# Autodesk Inventor assembly: Assembly_for_print
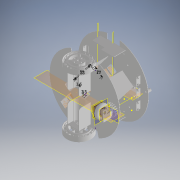
[picture p0: Inventor's stored thumbnail of the model, 180x180]
Saved by Autodesk Inventor 2020 (Build 240168000, 168)
## iProperties
Created: 2020-10-03
Part Number: Assembly_for_print
Document SubType Name: Assembly
Designer: Sičaja
Author: Sičaja
## Documents named in this file (7)
- C:\Users\Sicaja\Documents\Projects\3D Drawings\Inventor_draws\Robocup\Inverntor_parts_for_print\Assembly_for_print.iam
- C:\Users\Sicaja\Documents\Projects\3D Drawings\Inventor_draws\Robocup\Inverntor_parts_for_print\DropMechanism_v.2.0.ipt
- C:\Users\Sicaja\Documents\Projects\3D Drawings\Inventor_draws\Robocup\Inverntor_parts_for_print\KonstrukcijaDonjiDio_v.1.1.ipt
- C:\Users\Sicaja\Documents\Projects\3D Drawings\Inventor_draws\Robocup\Inverntor_parts_for_print\Gornja_konstrukcija_s_držačima_assembly_converted.ipt
- C:\Users\Sicaja\Documents\Projects\3D Drawings\Inventor_draws\Robocup\Inverntor_parts_for_print\Kotač_v.2.0.ipt
- C:\Users\Sicaja\Documents\Projects\3D Drawings\Inventor_draws\Robocup\Inverntor_parts_for_print\DrzacZaPrednjiKotač_v.1.0.ipt
- C:\Users\Sicaja\Documents\Projects\3D Drawings\Inventor_draws\Robocup\Inverntor_parts_for_print\PrednjiKotač_635z_lezaj_v.2.0.ipt
## Components (7 placed, 6 different names)
1. DropMechanism_v.2.0:1 — Mate:1, Mate:2, Flush:1
2. KonstrukcijaDonjiDio_v.1.1:1 — Mate:1, Mate:2, Flush:1, Mate:3, Mate:4, Insert:1, Insert:2, Mate:14, Insert:3, Mate:15, Insert:5, Insert:6
3. Gornja_konstrukcija_s_držačima_assembly_converted:1 — Mate:3, Mate:4, Mate:15, Insert:5, Insert:6
4. Kotač_v.2.0:1 — Insert:1
5. Kotač_v.2.0:2 — Insert:2
6. DrzacZaPrednjiKotač_v.1.0:1 — Mate:14, Insert:3, Insert:4
7. PrednjiKotač_635z_lezaj_v.2.0:1 — Insert:4
## Relationships (13: Mate 6, Insert 6, Flush 1)
- Mate:1: DropMechanism_v.2.0:1 ↔ KonstrukcijaDonjiDio_v.1.1:1
- Mate:2 (6 mm): DropMechanism_v.2.0:1 ↔ KonstrukcijaDonjiDio_v.1.1:1
- Flush:1 (-12 mm): DropMechanism_v.2.0:1 ↔ KonstrukcijaDonjiDio_v.1.1:1
- Mate:3 (60 mm): KonstrukcijaDonjiDio_v.1.1:1 ↔ Gornja_konstrukcija_s_držačima_assembly_converted:1
- Mate:4: KonstrukcijaDonjiDio_v.1.1:1 ↔ Gornja_konstrukcija_s_držačima_assembly_converted:1
- Insert:1 (5 mm): KonstrukcijaDonjiDio_v.1.1:1 ↔ Kotač_v.2.0:1
- Insert:2 (5 mm): KonstrukcijaDonjiDio_v.1.1:1 ↔ Kotač_v.2.0:2
- Mate:14: KonstrukcijaDonjiDio_v.1.1:1 ↔ DrzacZaPrednjiKotač_v.1.0:1
- Insert:3: KonstrukcijaDonjiDio_v.1.1:1 ↔ DrzacZaPrednjiKotač_v.1.0:1
- Insert:4: DrzacZaPrednjiKotač_v.1.0:1 ↔ PrednjiKotač_635z_lezaj_v.2.0:1
- Mate:15 (60 mm): KonstrukcijaDonjiDio_v.1.1:1 ↔ Gornja_konstrukcija_s_držačima_assembly_converted:1
- Insert:5: KonstrukcijaDonjiDio_v.1.1:1 ↔ Gornja_konstrukcija_s_držačima_assembly_converted:1
- Insert:6: KonstrukcijaDonjiDio_v.1.1:1 ↔ Gornja_konstrukcija_s_držačima_assembly_converted:1
